# Autodesk Inventor assembly: Assembly2
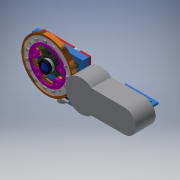
[picture p0: Inventor's stored thumbnail of the model, 180x180]
Saved by Autodesk Inventor 2017 (Build 210142000, 142)
## iProperties
Created: 2016-12-20
Part Number: Assembly2
Document SubType Name: Assembly
Designer: PLTW
Author: PLTW
## Documents named in this file (11)
- C:\Users\Roksbot\Documents\Inventor\PixyCam and Gimbal\Assembly2.iam
- C:\Users\Roksbot\Documents\Inventor\PixyCam and Gimbal\PixyCamKinda.ipt
- C:\Users\Roksbot\Documents\Inventor\PixyCam and Gimbal\focusSpacer.ipt
- C:\Users\Roksbot\Documents\Inventor\PixyCam and Gimbal\LEDRing.ipt
- C:\Users\Roksbot\Documents\Inventor\PixyCam and Gimbal\backCase.ipt
- C:\Users\Roksbot\Documents\Inventor\PixyCam and Gimbal\frontCase.ipt
- C:\Users\Roksbot\Documents\Inventor\PixyCam and Gimbal\Ring Front.ipt
- C:\Users\Roksbot\Documents\Inventor\PixyCam and Gimbal\Ring Holder.ipt
- C:\Users\Roksbot\Documents\Inventor\PixyCam and Gimbal\The Holdy Thing.ipt
- C:\Users\Roksbot\Documents\Inventor\PixyCam and Gimbal\servo arm.ipt
- C:\Users\Roksbot\Documents\Inventor\PixyCam and Gimbal\OtherCamera.ipt
## Components (10 placed, 10 different names)
1. PixyCamKinda:1 — Insert:1, Insert:2, Flush:1, Flush:2, Flush:3, Flush:4, Mate:2
2. focusSpacer:1 — Insert:1
3. LEDRing:1 — Insert:2, Flush:6, Flush:7
4. backCase:1 — Flush:1, Flush:2, Flush:5
5. frontCase:1 — Flush:3, Flush:4, Flush:5, Flush:11, Flush:12, Mate:1, Mate:3, Flush:13, Flush:14
6. Ring Front:1 — Flush:6, Flush:7, Flush:8, Flush:9
7. Ring Holder:1 — Flush:8, Flush:9, Flush:10, Tangent:1
8. The Holdy Thing:1 — Flush:10, Flush:11, Flush:12
9. servo arm:1 — Mate:1, Mate:2, Mate:3
10. OtherCamera:1 — Tangent:1, Flush:13, Flush:14
## Relationships (20: Flush 14, Mate 3, Insert 2, Tangent 1)
- Insert:1: PixyCamKinda:1 ↔ focusSpacer:1
- Insert:2: PixyCamKinda:1 ↔ LEDRing:1
- Flush:1: PixyCamKinda:1 ↔ backCase:1
- Flush:2: PixyCamKinda:1 ↔ backCase:1
- Flush:3: PixyCamKinda:1 ↔ frontCase:1
- Flush:4: PixyCamKinda:1 ↔ frontCase:1
- Flush:5: backCase:1 ↔ frontCase:1
- Flush:6: LEDRing:1 ↔ Ring Front:1
- Flush:7: LEDRing:1 ↔ Ring Front:1
- Flush:8: Ring Front:1 ↔ Ring Holder:1
- Flush:9: Ring Front:1 ↔ Ring Holder:1
- Flush:10: Ring Holder:1 ↔ The Holdy Thing:1
- Flush:11: frontCase:1 ↔ The Holdy Thing:1
- Flush:12: frontCase:1 ↔ The Holdy Thing:1
- Mate:1 (6.35 mm): frontCase:1 ↔ servo arm:1
- Mate:2: PixyCamKinda:1 ↔ servo arm:1
- Mate:3 (3.81 mm): frontCase:1 ↔ servo arm:1
- Tangent:1 (2.54 mm): Ring Holder:1 ↔ OtherCamera:1
- Flush:13: frontCase:1 ↔ OtherCamera:1
- Flush:14: frontCase:1 ↔ OtherCamera:1
